# Autodesk Inventor assembly: V5Climb
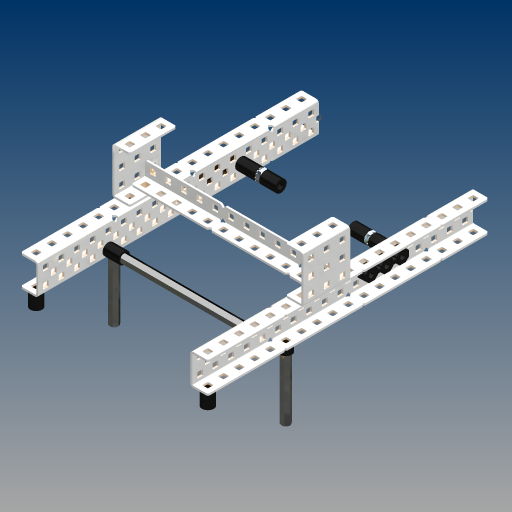
[picture p0: Inventor's stored thumbnail of the model, 512x512]
Saved by Autodesk Inventor 2023 (Build 270158000, 158)
## iProperties
Created: 2024-02-14
Part Number: V5Climb
Document SubType Name: Assembly
Designer: eddie
Author: eddie
## Documents named in this file (15)
- C:\Users\eddie\Documents\81208X-Over-Under-CAD\Custom-parts\V5Climb.iam
- C:\Users\eddie\Documents\81208X-Over-Under-CAD\VEX-CAD-Inventor-1.4.0\Structure\C Channel\Aluminum 1x2x1\Alu C 1x2x1x18.ipt
- C:\Users\eddie\Documents\81208X-Over-Under-CAD\VEX-CAD-Inventor-1.4.0\Structure\Angle\Aluminum\1x1\Alu Angle 1x1x12.ipt
- C:\Users\eddie\Documents\81208X-Over-Under-CAD\VEX-CAD-Inventor-1.4.0\Structure\C Channel\Aluminum 1x3x1\Alu C 1x3x1x3.ipt
- C:\Users\eddie\Documents\81208X-Over-Under-CAD\VEX-CAD-Inventor-1.4.0\Motion\Spacers\Spacer Nylon .375 OD\NSpacer .375 OD x .500.ipt
- C:\Users\eddie\Documents\81208X-Over-Under-CAD\VEX-CAD-Inventor-1.4.0\Motion\Spacers\Spacer Nylon .375 OD.ipt
- C:\Users\eddie\Documents\81208X-Over-Under-CAD\VEX-CAD-Inventor-1.4.0\Structure\Standoff\Standoff 4.00.ipt
- C:\Users\eddie\Documents\81208X-Over-Under-CAD\VEX-CAD-Inventor-1.4.0\Structure\Standoff.ipt
- C:\Users\eddie\Documents\81208X-Over-Under-CAD\VEX-CAD-Inventor-1.4.0\Motion\Spacers\Spacer Nylon .500 OD\NSpacer White .500 OD x .375.ipt
- C:\Users\eddie\Documents\81208X-Over-Under-CAD\VEX-CAD-Inventor-1.4.0\Motion\Spacers\Spacer Nylon .500 OD.ipt
- C:\Users\eddie\Documents\81208X-Over-Under-CAD\VEX-CAD-Inventor-1.4.0\Motion\Shaft LS\Bearing Flat.ipt
- C:\Users\eddie\Documents\81208X-Over-Under-CAD\VEX-CAD-Inventor-1.4.0\Motion\Spacers\Spacer Nylon .375 OD\NSpacer .375 OD x .375.ipt
- C:\Users\eddie\Documents\81208X-Over-Under-CAD\VEX-CAD-Inventor-1.4.0\Motion\Spacers\Spacer Nylon .375 OD\NSpacer .375 OD x .250.ipt
- C:\Users\eddie\Documents\81208X-Over-Under-CAD\VEX-CAD-Inventor-1.4.0\Structure\Hardware\Nut Keps.ipt
- C:\Users\eddie\Documents\81208X-Over-Under-CAD\VEX-CAD-Inventor-1.4.0\Structure\Standoff\Standoff 2.00.ipt
## Components (24 placed, 11 different names)
1. Alu C 1x2x1x18:1 — Insert:1, Insert:5, Insert:9, Insert:14, Insert:18, Insert:20
2. Alu C 1x2x1x18:2 — Insert:2, Insert:8, Insert:10, Insert:19, Insert:21
3. Alu Angle 1x1x12:1 — Insert:3, Insert:4
4. Alu C 1x3x1x3:1 — Insert:2, Insert:4
5. Alu C 1x3x1x3:2 — Insert:1, Insert:3
6. NSpacer .375 OD x .500:1 — Insert:5, Insert:6
7. Standoff 4.00:1 — Insert:6, Insert:7
8. NSpacer White .500 OD x .375:1 — Insert:7
9. Bearing Flat:1 — Insert:8
10. Bearing Flat:2 — Insert:9
11. NSpacer .375 OD x .375:2 — Insert:10, Insert:11
12. NSpacer .375 OD x .250:3 — Insert:11, Insert:12
13. NSpacer .375 OD x .500:4 — Insert:17
14. Nut Keps:1 — Insert:12, Insert:13
15. Nut Keps:2 — Insert:16, Insert:17
16. NSpacer .375 OD x .500:5 — Insert:13
17. NSpacer .375 OD x .375:6 — Insert:14, Insert:15
18. NSpacer .375 OD x .250:7 — Insert:15, Insert:16
19. NSpacer .375 OD x .500:8 — Insert:18
20. NSpacer .375 OD x .500:9 — Insert:19
21. NSpacer .375 OD x .250:10 — Insert:21, Insert:22
22. NSpacer .375 OD x .250:11 — Insert:20, Insert:23
23. Standoff 2.00:2 — Insert:22
24. Standoff 2.00:3 — Insert:23
## Relationships (23: Insert 23)
- Insert:1: Alu C 1x2x1x18:1 ↔ Alu C 1x3x1x3:2
- Insert:2: Alu C 1x2x1x18:2 ↔ Alu C 1x3x1x3:1
- Insert:3: Alu Angle 1x1x12:1 ↔ Alu C 1x3x1x3:2
- Insert:4: Alu Angle 1x1x12:1 ↔ Alu C 1x3x1x3:1
- Insert:5: Alu C 1x2x1x18:1 ↔ NSpacer .375 OD x .500:1
- Insert:6: NSpacer .375 OD x .500:1 ↔ Standoff 4.00:1
- Insert:7: Standoff 4.00:1 ↔ NSpacer White .500 OD x .375:1
- Insert:8: Alu C 1x2x1x18:2 ↔ Bearing Flat:1
- Insert:9: Alu C 1x2x1x18:1 ↔ Bearing Flat:2
- Insert:10: Alu C 1x2x1x18:2 ↔ NSpacer .375 OD x .375:2
- Insert:11: NSpacer .375 OD x .375:2 ↔ NSpacer .375 OD x .250:3
- Insert:12: NSpacer .375 OD x .250:3 ↔ Nut Keps:1
- Insert:13: Nut Keps:1 ↔ NSpacer .375 OD x .500:5
- Insert:14: Alu C 1x2x1x18:1 ↔ NSpacer .375 OD x .375:6
- Insert:15: NSpacer .375 OD x .375:6 ↔ NSpacer .375 OD x .250:7
- Insert:16: Nut Keps:2 ↔ NSpacer .375 OD x .250:7
- Insert:17: NSpacer .375 OD x .500:4 ↔ Nut Keps:2
- Insert:18: Alu C 1x2x1x18:1 ↔ NSpacer .375 OD x .500:8
- Insert:19: Alu C 1x2x1x18:2 ↔ NSpacer .375 OD x .500:9
- Insert:20: Alu C 1x2x1x18:1 ↔ NSpacer .375 OD x .250:11
- Insert:21: Alu C 1x2x1x18:2 ↔ NSpacer .375 OD x .250:10
- Insert:22: NSpacer .375 OD x .250:10 ↔ Standoff 2.00:2
- Insert:23: NSpacer .375 OD x .250:11 ↔ Standoff 2.00:3
